# Autodesk Inventor assembly: RD53A-2x2_hdi_pickup_tool_assembly_v2
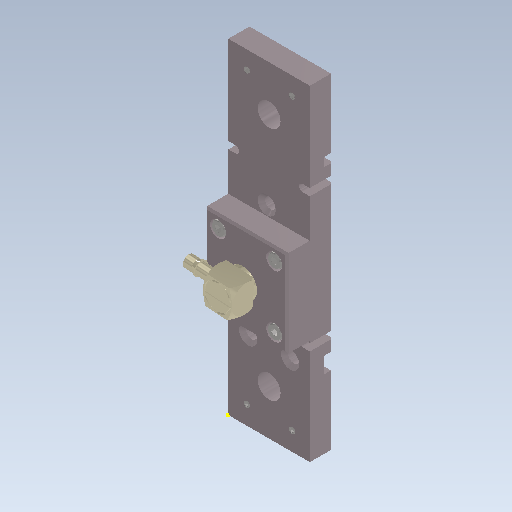
[picture p0: Inventor's stored thumbnail of the model, 512x512]
Saved by Autodesk Inventor 2021 (Build 250183000, 183)
## iProperties
Created: 2021-08-27
Part Number: RD53A-2x2_hdi_pickup_tool_assembly_v2
Document SubType Name: Assembly
Designer: mjones
Author: mjones
## Documents named in this file (6)
- C:\Users\mjones\Documents\CMS\Phase2\Inventor\RD53A-2x2_hdi_pickup_tool_assembly_v2.iam
- C:\Users\mjones\Documents\CMS\Phase2\Inventor\RD53A-2x2_hdi_pickup_tool_v2.ipt
- C:\Users\mjones\Documents\CMS\Phase2\Inventor\RD53A-2x2_hdi_vacuum_cover_v2.ipt
- C:\Users\mjones\Documents\CMS\Phase2\Inventor\2844K730_NICKEL-PLTD BRASS BARBED VACUUM TUBE FITTING.ipt
- C:\Users\mjones\Documents\CMS\Phase2\Inventor\91292A832_TYPE 18-8 SS SOCKET HEAD CAP SCREW.ipt
- C:\Users\mjones\Documents\CMS\Phase2\Inventor\92605A912_STAINLESS STEEL FLAT-TIP SET SCREW.ipt
## Components (11 placed, 5 different names)
1. RD53A-2x2_hdi_pickup_tool_v2:1 — Mate:1, Insert:7, Insert:8, Insert:9, Insert:10, Insert:11, Insert:12
2. RD53A-2x2_hdi_vacuum_cover_v2:1 — Insert:2, Insert:3, Insert:4, Insert:5, Insert:6, Insert:7, Insert:8
3. 2844K730_NICKEL-PLTD BRASS BARBED VACUUM TUBE FITTING:1 — Insert:2
4. 91292A832_TYPE 18-8 SS SOCKET HEAD CAP SCREW:1 — Insert:3
5. 91292A832_TYPE 18-8 SS SOCKET HEAD CAP SCREW:2 — Insert:4
6. 91292A832_TYPE 18-8 SS SOCKET HEAD CAP SCREW:3 — Insert:6
7. 91292A832_TYPE 18-8 SS SOCKET HEAD CAP SCREW:4 — Insert:5
8. 92605A912_STAINLESS STEEL FLAT-TIP SET SCREW:1 — Insert:9
9. 92605A912_STAINLESS STEEL FLAT-TIP SET SCREW:2 — Insert:10
10. 92605A912_STAINLESS STEEL FLAT-TIP SET SCREW:3 — Insert:11
11. 92605A912_STAINLESS STEEL FLAT-TIP SET SCREW:4 — Insert:12
## Relationships (12: Insert 11, Mate 1)
- Insert:2: RD53A-2x2_hdi_vacuum_cover_v2:1 ↔ 2844K730_NICKEL-PLTD BRASS BARBED VACUUM TUBE FITTING:1
- Insert:3: RD53A-2x2_hdi_vacuum_cover_v2:1 ↔ 91292A832_TYPE 18-8 SS SOCKET HEAD CAP SCREW:1
- Insert:4: RD53A-2x2_hdi_vacuum_cover_v2:1 ↔ 91292A832_TYPE 18-8 SS SOCKET HEAD CAP SCREW:2
- Insert:5: RD53A-2x2_hdi_vacuum_cover_v2:1 ↔ 91292A832_TYPE 18-8 SS SOCKET HEAD CAP SCREW:4
- Insert:6: RD53A-2x2_hdi_vacuum_cover_v2:1 ↔ 91292A832_TYPE 18-8 SS SOCKET HEAD CAP SCREW:3
- Mate:1: RD53A-2x2_hdi_pickup_tool_v2:1
- Insert:7: RD53A-2x2_hdi_pickup_tool_v2:1 ↔ RD53A-2x2_hdi_vacuum_cover_v2:1
- Insert:8: RD53A-2x2_hdi_pickup_tool_v2:1 ↔ RD53A-2x2_hdi_vacuum_cover_v2:1
- Insert:9: RD53A-2x2_hdi_pickup_tool_v2:1 ↔ 92605A912_STAINLESS STEEL FLAT-TIP SET SCREW:1
- Insert:10: RD53A-2x2_hdi_pickup_tool_v2:1 ↔ 92605A912_STAINLESS STEEL FLAT-TIP SET SCREW:2
- Insert:11: RD53A-2x2_hdi_pickup_tool_v2:1 ↔ 92605A912_STAINLESS STEEL FLAT-TIP SET SCREW:3
- Insert:12: RD53A-2x2_hdi_pickup_tool_v2:1 ↔ 92605A912_STAINLESS STEEL FLAT-TIP SET SCREW:4
